# Autodesk Inventor assembly: Stadio8
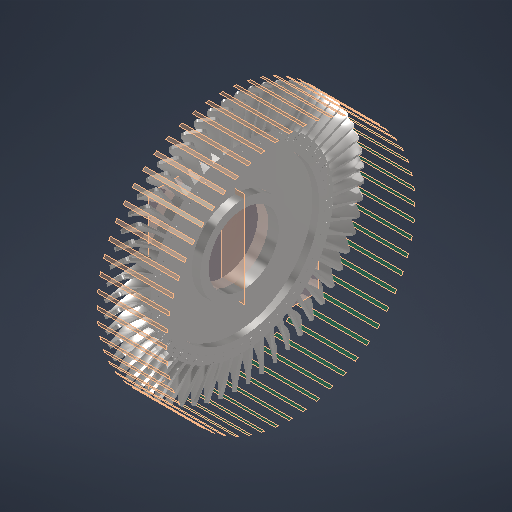
[picture p0: Inventor's stored thumbnail of the model, 512x512]
Saved by Autodesk Inventor 2026.2 (Build 302298010, 298A)
## iProperties
Created: 2026-04-24
Part Number: Stadio8
Document SubType Name: Assembly
Designer: Yan
Author: Yan
## Documents named in this file (3)
- C:\Users\Yan\Desktop\Turbina\Stadio8.iam
- C:\Users\Yan\Desktop\Turbina\DiscoPaleStadio8-DimensioniAprossimate.ipt
- C:\Users\Yan\Desktop\Turbina\PalaStadio8.ipt
## Components (57 placed, 2 different names)
1. DiscoPaleStadio8-DimensioniAprossimate:1 — Mate:1, Mate:2, Mate:3, Mate:4, Mate:5, Mate:6, Mate:7, Mate:8, Mate:9, Mate:10, Mate:11, Mate:12, Mate:13, Mate:14, Mate:15, Mate:16, Mate:17, Mate:18, Mate:19, Mate:20, Mate:21, Mate:22, Mate:23, Mate:24, Mate:25, Mate:26, Mate:27, Mate:28, Mate:29, Mate:30, Mate:31, Mate:32, Mate:33, Mate:34, Mate:35, Mate:36, Mate:37, Mate:38, Mate:39, Mate:40, Mate:41, Mate:42, Mate:43, Mate:44, Mate:45, Mate:46, Mate:47, Mate:48, Mate:49, Mate:50, Mate:51, Mate:52, Mate:53, Mate:54, Mate:55, Mate:56, Mate:57, Mate:58, Mate:59, Mate:60, Mate:62, Mate:63, Mate:64, Mate:65, Mate:66, Mate:67, Mate:68, Mate:69, Mate:70, Mate:71, Mate:72, Mate:73, Mate:74, Mate:75, Mate:76, Mate:77, Mate:78, Mate:79, Mate:80, Mate:81, Mate:82, Mate:83, Mate:84, Mate:85, Mate:86, Mate:87, Mate:88, Mate:89, Mate:90, Mate:91, Mate:92, Mate:93, Mate:94, Mate:95, Mate:96, Mate:97, Mate:98, Mate:99, Mate:100, Mate:101, Mate:102, Mate:103, Mate:104, Mate:105, Mate:106, Mate:107, Mate:108, Mate:109, Mate:110, Mate:111, Mate:112, Flush:1, Flush:2, Flush:3, Flush:4, Flush:5, Flush:6, Flush:7, Flush:8, Flush:9, Flush:10, Flush:11, Flush:12, Flush:13, Flush:14, Flush:15, Flush:16, Flush:17, Flush:18, Flush:19, Flush:20, Flush:21, Flush:22, Flush:23, Flush:24, Flush:25, Flush:26, Flush:27, Flush:28, Flush:29, Flush:30, Flush:31, Flush:32, Flush:33, Flush:34, Flush:35, Flush:36, Flush:37, Flush:38, Flush:39, Flush:40, Flush:41, Flush:42, Flush:43, Flush:44, Flush:45, Flush:46, Flush:47, Flush:48, Flush:49, Flush:50, Flush:51, Flush:52, Flush:53, Flush:54, Flush:55, Flush:56
2. PalaStadio8:1 — Mate:1, Mate:59, Flush:42
3. PalaStadio8:2 — Mate:2, Mate:58, Flush:43
4. PalaStadio8:3 — Mate:3, Mate:57, Flush:44
5. PalaStadio8:4 — Mate:4, Mate:56, Flush:45
6. PalaStadio8:5 — Mate:5, Mate:55, Flush:46
7. PalaStadio8:6 — Mate:6, Mate:54, Flush:47
8. PalaStadio8:7 — Mate:7, Mate:53, Flush:48
9. PalaStadio8:8 — Mate:8, Mate:52, Flush:49
10. PalaStadio8:9 — Mate:9, Mate:51, Flush:50
11. PalaStadio8:10 — Mate:10, Mate:50, Flush:51
12. PalaStadio8:11 — Mate:11, Mate:49, Flush:52
13. PalaStadio8:12 — Mate:12, Mate:48, Flush:53
14. PalaStadio8:13 — Mate:13, Mate:47, Flush:54
15. PalaStadio8:14 — Mate:14, Mate:46, Flush:55
16. PalaStadio8:15 — Mate:15, Mate:45, Flush:56
17. PalaStadio8:16 — Mate:16, Mate:44, Flush:2
18. PalaStadio8:17 — Mate:17, Mate:43, Flush:1
19. PalaStadio8:18 — Mate:18, Mate:42, Flush:3
20. PalaStadio8:19 — Mate:19, Mate:41, Flush:4
21. PalaStadio8:20 — Mate:20, Mate:40, Flush:5
22. PalaStadio8:21 — Mate:30, Mate:32, Flush:15
23. PalaStadio8:22 — Mate:29, Mate:31, Flush:14
24. PalaStadio8:23 — Mate:28, Mate:33, Flush:13
25. PalaStadio8:24 — Mate:27, Mate:60, Flush:12
26. PalaStadio8:25 — Mate:26, Mate:34, Flush:11
27. PalaStadio8:26 — Mate:25, Mate:35, Flush:10
28. PalaStadio8:27 — Mate:24, Mate:36, Flush:9
29. PalaStadio8:28 — Mate:23, Mate:37, Flush:8
30. PalaStadio8:29 — Mate:22, Mate:38, Flush:7
31. PalaStadio8:30 — Mate:21, Mate:39, Flush:6
32. PalaStadio8:31 — Mate:62, Mate:111, Flush:17
33. PalaStadio8:32 — Mate:64, Mate:112, Flush:18
34. PalaStadio8:33 — Mate:65, Mate:109, Flush:19
35. PalaStadio8:34 — Mate:66, Mate:108, Flush:20
36. PalaStadio8:35 — Mate:67, Mate:107, Flush:21
37. PalaStadio8:36 — Mate:68, Mate:106, Flush:22
38. PalaStadio8:37 — Mate:69, Mate:105, Flush:23
39. PalaStadio8:38 — Mate:70, Mate:104, Flush:24
40. PalaStadio8:39 — Mate:71, Mate:103, Flush:25
41. PalaStadio8:40 — Mate:63, Mate:110, Flush:16
42. PalaStadio8:41 — Mate:81, Mate:94, Flush:35
43. PalaStadio8:42 — Mate:80, Mate:95, Flush:34
44. PalaStadio8:43 — Mate:79, Mate:96, Flush:33
45. PalaStadio8:44 — Mate:78, Mate:97, Flush:32
46. PalaStadio8:45 — Mate:77, Mate:98, Flush:31
47. PalaStadio8:46 — Mate:76, Mate:99, Flush:30
48. PalaStadio8:47 — Mate:75, Mate:100, Flush:29
49. PalaStadio8:48 — Mate:74, Flush:28
50. PalaStadio8:49 — Mate:73, Mate:101, Flush:27
51. PalaStadio8:50 — Mate:72, Mate:102, Flush:26
52. PalaStadio8:51 — Mate:87, Mate:88, Flush:41
53. PalaStadio8:52 — Mate:86, Mate:89, Flush:40
54. PalaStadio8:53 — Mate:85, Mate:90, Flush:39
55. PalaStadio8:54 — Mate:84, Mate:91, Flush:38
56. PalaStadio8:55 — Mate:83, Mate:92, Flush:37
57. PalaStadio8:56 — Mate:82, Mate:93, Flush:36
## Relationships (167: Mate 111, Flush 56)
- Mate:1: DiscoPaleStadio8-DimensioniAprossimate:1 ↔ PalaStadio8:1
- Mate:2: DiscoPaleStadio8-DimensioniAprossimate:1 ↔ PalaStadio8:2
- Mate:3: DiscoPaleStadio8-DimensioniAprossimate:1 ↔ PalaStadio8:3
- Mate:4: DiscoPaleStadio8-DimensioniAprossimate:1 ↔ PalaStadio8:4
- Mate:5: DiscoPaleStadio8-DimensioniAprossimate:1 ↔ PalaStadio8:5
- Mate:6: DiscoPaleStadio8-DimensioniAprossimate:1 ↔ PalaStadio8:6
- Mate:7: DiscoPaleStadio8-DimensioniAprossimate:1 ↔ PalaStadio8:7
- Mate:8: DiscoPaleStadio8-DimensioniAprossimate:1 ↔ PalaStadio8:8
- Mate:9: DiscoPaleStadio8-DimensioniAprossimate:1 ↔ PalaStadio8:9
- Mate:10: DiscoPaleStadio8-DimensioniAprossimate:1 ↔ PalaStadio8:10
- Mate:11: DiscoPaleStadio8-DimensioniAprossimate:1 ↔ PalaStadio8:11
- Mate:12: DiscoPaleStadio8-DimensioniAprossimate:1 ↔ PalaStadio8:12
- Mate:13: DiscoPaleStadio8-DimensioniAprossimate:1 ↔ PalaStadio8:13
- Mate:14: DiscoPaleStadio8-DimensioniAprossimate:1 ↔ PalaStadio8:14
- Mate:15: DiscoPaleStadio8-DimensioniAprossimate:1 ↔ PalaStadio8:15
- Mate:16: DiscoPaleStadio8-DimensioniAprossimate:1 ↔ PalaStadio8:16
- Mate:17: DiscoPaleStadio8-DimensioniAprossimate:1 ↔ PalaStadio8:17
- Mate:18: DiscoPaleStadio8-DimensioniAprossimate:1 ↔ PalaStadio8:18
- Mate:19: DiscoPaleStadio8-DimensioniAprossimate:1 ↔ PalaStadio8:19
- Mate:20: DiscoPaleStadio8-DimensioniAprossimate:1 ↔ PalaStadio8:20
- Mate:21: DiscoPaleStadio8-DimensioniAprossimate:1 ↔ PalaStadio8:30
- Mate:22: DiscoPaleStadio8-DimensioniAprossimate:1 ↔ PalaStadio8:29
- Mate:23: DiscoPaleStadio8-DimensioniAprossimate:1 ↔ PalaStadio8:28
- Mate:24: DiscoPaleStadio8-DimensioniAprossimate:1 ↔ PalaStadio8:27
- Mate:25: DiscoPaleStadio8-DimensioniAprossimate:1 ↔ PalaStadio8:26
- Mate:26: DiscoPaleStadio8-DimensioniAprossimate:1 ↔ PalaStadio8:25
- Mate:27: DiscoPaleStadio8-DimensioniAprossimate:1 ↔ PalaStadio8:24
- Mate:28: DiscoPaleStadio8-DimensioniAprossimate:1 ↔ PalaStadio8:23
- Mate:29: DiscoPaleStadio8-DimensioniAprossimate:1 ↔ PalaStadio8:22
- Mate:30: DiscoPaleStadio8-DimensioniAprossimate:1 ↔ PalaStadio8:21
- Mate:31: DiscoPaleStadio8-DimensioniAprossimate:1 ↔ PalaStadio8:22
- Mate:32: DiscoPaleStadio8-DimensioniAprossimate:1 ↔ PalaStadio8:21
- Mate:33: DiscoPaleStadio8-DimensioniAprossimate:1 ↔ PalaStadio8:23
- Mate:34: DiscoPaleStadio8-DimensioniAprossimate:1 ↔ PalaStadio8:25
- Mate:35: DiscoPaleStadio8-DimensioniAprossimate:1 ↔ PalaStadio8:26
- Mate:36: DiscoPaleStadio8-DimensioniAprossimate:1 ↔ PalaStadio8:27
- Mate:37: DiscoPaleStadio8-DimensioniAprossimate:1 ↔ PalaStadio8:28
- Mate:38: DiscoPaleStadio8-DimensioniAprossimate:1 ↔ PalaStadio8:29
- Mate:39: DiscoPaleStadio8-DimensioniAprossimate:1 ↔ PalaStadio8:30
- Mate:40: DiscoPaleStadio8-DimensioniAprossimate:1 ↔ PalaStadio8:20
- Mate:41: DiscoPaleStadio8-DimensioniAprossimate:1 ↔ PalaStadio8:19
- Mate:42: DiscoPaleStadio8-DimensioniAprossimate:1 ↔ PalaStadio8:18
- Mate:43: DiscoPaleStadio8-DimensioniAprossimate:1 ↔ PalaStadio8:17
- Mate:44: DiscoPaleStadio8-DimensioniAprossimate:1 ↔ PalaStadio8:16
- Mate:45: DiscoPaleStadio8-DimensioniAprossimate:1 ↔ PalaStadio8:15
- Mate:46: DiscoPaleStadio8-DimensioniAprossimate:1 ↔ PalaStadio8:14
- Mate:47: DiscoPaleStadio8-DimensioniAprossimate:1 ↔ PalaStadio8:13
- Mate:48: DiscoPaleStadio8-DimensioniAprossimate:1 ↔ PalaStadio8:12
- Mate:49: DiscoPaleStadio8-DimensioniAprossimate:1 ↔ PalaStadio8:11
- Mate:50: DiscoPaleStadio8-DimensioniAprossimate:1 ↔ PalaStadio8:10
- Mate:51: DiscoPaleStadio8-DimensioniAprossimate:1 ↔ PalaStadio8:9
- Mate:52: DiscoPaleStadio8-DimensioniAprossimate:1 ↔ PalaStadio8:8
- Mate:53: DiscoPaleStadio8-DimensioniAprossimate:1 ↔ PalaStadio8:7
- Mate:54: DiscoPaleStadio8-DimensioniAprossimate:1 ↔ PalaStadio8:6
- Mate:55: DiscoPaleStadio8-DimensioniAprossimate:1 ↔ PalaStadio8:5
- Mate:56: DiscoPaleStadio8-DimensioniAprossimate:1 ↔ PalaStadio8:4
- Mate:57: DiscoPaleStadio8-DimensioniAprossimate:1 ↔ PalaStadio8:3
- Mate:58: DiscoPaleStadio8-DimensioniAprossimate:1 ↔ PalaStadio8:2
- Mate:59: DiscoPaleStadio8-DimensioniAprossimate:1 ↔ PalaStadio8:1
- Mate:60: DiscoPaleStadio8-DimensioniAprossimate:1 ↔ PalaStadio8:24
- Mate:62: DiscoPaleStadio8-DimensioniAprossimate:1 ↔ PalaStadio8:31
- Mate:63: DiscoPaleStadio8-DimensioniAprossimate:1 ↔ PalaStadio8:40
- Mate:64: DiscoPaleStadio8-DimensioniAprossimate:1 ↔ PalaStadio8:32
- Mate:65: DiscoPaleStadio8-DimensioniAprossimate:1 ↔ PalaStadio8:33
- Mate:66: DiscoPaleStadio8-DimensioniAprossimate:1 ↔ PalaStadio8:34
- Mate:67: DiscoPaleStadio8-DimensioniAprossimate:1 ↔ PalaStadio8:35
- Mate:68: DiscoPaleStadio8-DimensioniAprossimate:1 ↔ PalaStadio8:36
- Mate:69: DiscoPaleStadio8-DimensioniAprossimate:1 ↔ PalaStadio8:37
- Mate:70: DiscoPaleStadio8-DimensioniAprossimate:1 ↔ PalaStadio8:38
- Mate:71: DiscoPaleStadio8-DimensioniAprossimate:1 ↔ PalaStadio8:39
- Mate:72: DiscoPaleStadio8-DimensioniAprossimate:1 ↔ PalaStadio8:50
- Mate:73: DiscoPaleStadio8-DimensioniAprossimate:1 ↔ PalaStadio8:49
- Mate:74: DiscoPaleStadio8-DimensioniAprossimate:1 ↔ PalaStadio8:48
- Mate:75: DiscoPaleStadio8-DimensioniAprossimate:1 ↔ PalaStadio8:47
- Mate:76: DiscoPaleStadio8-DimensioniAprossimate:1 ↔ PalaStadio8:46
- Mate:77: DiscoPaleStadio8-DimensioniAprossimate:1 ↔ PalaStadio8:45
- Mate:78: DiscoPaleStadio8-DimensioniAprossimate:1 ↔ PalaStadio8:44
- Mate:79: DiscoPaleStadio8-DimensioniAprossimate:1 ↔ PalaStadio8:43
- Mate:80: DiscoPaleStadio8-DimensioniAprossimate:1 ↔ PalaStadio8:42
- Mate:81: DiscoPaleStadio8-DimensioniAprossimate:1 ↔ PalaStadio8:41
- Mate:82: DiscoPaleStadio8-DimensioniAprossimate:1 ↔ PalaStadio8:56
- Mate:83: DiscoPaleStadio8-DimensioniAprossimate:1 ↔ PalaStadio8:55
- Mate:84: DiscoPaleStadio8-DimensioniAprossimate:1 ↔ PalaStadio8:54
- Mate:85: DiscoPaleStadio8-DimensioniAprossimate:1 ↔ PalaStadio8:53
- Mate:86: DiscoPaleStadio8-DimensioniAprossimate:1 ↔ PalaStadio8:52
- Mate:87: DiscoPaleStadio8-DimensioniAprossimate:1 ↔ PalaStadio8:51
- Mate:88: DiscoPaleStadio8-DimensioniAprossimate:1 ↔ PalaStadio8:51
- Mate:89: DiscoPaleStadio8-DimensioniAprossimate:1 ↔ PalaStadio8:52
- Mate:90: DiscoPaleStadio8-DimensioniAprossimate:1 ↔ PalaStadio8:53
- Mate:91: DiscoPaleStadio8-DimensioniAprossimate:1 ↔ PalaStadio8:54
- Mate:92: DiscoPaleStadio8-DimensioniAprossimate:1 ↔ PalaStadio8:55
- Mate:93: DiscoPaleStadio8-DimensioniAprossimate:1 ↔ PalaStadio8:56
- Mate:94: DiscoPaleStadio8-DimensioniAprossimate:1 ↔ PalaStadio8:41
- Mate:95: DiscoPaleStadio8-DimensioniAprossimate:1 ↔ PalaStadio8:42
- Mate:96: DiscoPaleStadio8-DimensioniAprossimate:1 ↔ PalaStadio8:43
- Mate:97: DiscoPaleStadio8-DimensioniAprossimate:1 ↔ PalaStadio8:44
- Mate:98: DiscoPaleStadio8-DimensioniAprossimate:1 ↔ PalaStadio8:45
- Mate:99: DiscoPaleStadio8-DimensioniAprossimate:1 ↔ PalaStadio8:46
- Mate:100: DiscoPaleStadio8-DimensioniAprossimate:1 ↔ PalaStadio8:47
- Mate:101: DiscoPaleStadio8-DimensioniAprossimate:1 ↔ PalaStadio8:49
- Mate:102: DiscoPaleStadio8-DimensioniAprossimate:1 ↔ PalaStadio8:50
- Mate:103: DiscoPaleStadio8-DimensioniAprossimate:1 ↔ PalaStadio8:39
- Mate:104: DiscoPaleStadio8-DimensioniAprossimate:1 ↔ PalaStadio8:38
- Mate:105: DiscoPaleStadio8-DimensioniAprossimate:1 ↔ PalaStadio8:37
- Mate:106: DiscoPaleStadio8-DimensioniAprossimate:1 ↔ PalaStadio8:36
- Mate:107: DiscoPaleStadio8-DimensioniAprossimate:1 ↔ PalaStadio8:35
- Mate:108: DiscoPaleStadio8-DimensioniAprossimate:1 ↔ PalaStadio8:34
- Mate:109: DiscoPaleStadio8-DimensioniAprossimate:1 ↔ PalaStadio8:33
- Mate:110: DiscoPaleStadio8-DimensioniAprossimate:1 ↔ PalaStadio8:40
- Mate:111: DiscoPaleStadio8-DimensioniAprossimate:1 ↔ PalaStadio8:31
- Mate:112: DiscoPaleStadio8-DimensioniAprossimate:1 ↔ PalaStadio8:32
- Flush:1: DiscoPaleStadio8-DimensioniAprossimate:1 ↔ PalaStadio8:17
- Flush:2: DiscoPaleStadio8-DimensioniAprossimate:1 ↔ PalaStadio8:16
- Flush:3: DiscoPaleStadio8-DimensioniAprossimate:1 ↔ PalaStadio8:18
- Flush:4: DiscoPaleStadio8-DimensioniAprossimate:1 ↔ PalaStadio8:19
- Flush:5: DiscoPaleStadio8-DimensioniAprossimate:1 ↔ PalaStadio8:20
- Flush:6: DiscoPaleStadio8-DimensioniAprossimate:1 ↔ PalaStadio8:30
- Flush:7: DiscoPaleStadio8-DimensioniAprossimate:1 ↔ PalaStadio8:29
- Flush:8: DiscoPaleStadio8-DimensioniAprossimate:1 ↔ PalaStadio8:28
- Flush:9: DiscoPaleStadio8-DimensioniAprossimate:1 ↔ PalaStadio8:27
- Flush:10: DiscoPaleStadio8-DimensioniAprossimate:1 ↔ PalaStadio8:26
- Flush:11: DiscoPaleStadio8-DimensioniAprossimate:1 ↔ PalaStadio8:25
- Flush:12: DiscoPaleStadio8-DimensioniAprossimate:1 ↔ PalaStadio8:24
- Flush:13: DiscoPaleStadio8-DimensioniAprossimate:1 ↔ PalaStadio8:23
- Flush:14: DiscoPaleStadio8-DimensioniAprossimate:1 ↔ PalaStadio8:22
- Flush:15: DiscoPaleStadio8-DimensioniAprossimate:1 ↔ PalaStadio8:21
- Flush:16: DiscoPaleStadio8-DimensioniAprossimate:1 ↔ PalaStadio8:40
- Flush:17: DiscoPaleStadio8-DimensioniAprossimate:1 ↔ PalaStadio8:31
- Flush:18: DiscoPaleStadio8-DimensioniAprossimate:1 ↔ PalaStadio8:32
- Flush:19: DiscoPaleStadio8-DimensioniAprossimate:1 ↔ PalaStadio8:33
- Flush:20: DiscoPaleStadio8-DimensioniAprossimate:1 ↔ PalaStadio8:34
- Flush:21: DiscoPaleStadio8-DimensioniAprossimate:1 ↔ PalaStadio8:35
- Flush:22: DiscoPaleStadio8-DimensioniAprossimate:1 ↔ PalaStadio8:36
- Flush:23: DiscoPaleStadio8-DimensioniAprossimate:1 ↔ PalaStadio8:37
- Flush:24: DiscoPaleStadio8-DimensioniAprossimate:1 ↔ PalaStadio8:38
- Flush:25: DiscoPaleStadio8-DimensioniAprossimate:1 ↔ PalaStadio8:39
- Flush:26: DiscoPaleStadio8-DimensioniAprossimate:1 ↔ PalaStadio8:50
- Flush:27: DiscoPaleStadio8-DimensioniAprossimate:1 ↔ PalaStadio8:49
- Flush:28: DiscoPaleStadio8-DimensioniAprossimate:1 ↔ PalaStadio8:48
- Flush:29: DiscoPaleStadio8-DimensioniAprossimate:1 ↔ PalaStadio8:47
- Flush:30: DiscoPaleStadio8-DimensioniAprossimate:1 ↔ PalaStadio8:46
- Flush:31: DiscoPaleStadio8-DimensioniAprossimate:1 ↔ PalaStadio8:45
- Flush:32: DiscoPaleStadio8-DimensioniAprossimate:1 ↔ PalaStadio8:44
- Flush:33: DiscoPaleStadio8-DimensioniAprossimate:1 ↔ PalaStadio8:43
- Flush:34: DiscoPaleStadio8-DimensioniAprossimate:1 ↔ PalaStadio8:42
- Flush:35: DiscoPaleStadio8-DimensioniAprossimate:1 ↔ PalaStadio8:41
- Flush:36: DiscoPaleStadio8-DimensioniAprossimate:1 ↔ PalaStadio8:56
- Flush:37: DiscoPaleStadio8-DimensioniAprossimate:1 ↔ PalaStadio8:55
- Flush:38: DiscoPaleStadio8-DimensioniAprossimate:1 ↔ PalaStadio8:54
- Flush:39: DiscoPaleStadio8-DimensioniAprossimate:1 ↔ PalaStadio8:53
- Flush:40: DiscoPaleStadio8-DimensioniAprossimate:1 ↔ PalaStadio8:52
- Flush:41: DiscoPaleStadio8-DimensioniAprossimate:1 ↔ PalaStadio8:51
- Flush:42: DiscoPaleStadio8-DimensioniAprossimate:1 ↔ PalaStadio8:1
- Flush:43: DiscoPaleStadio8-DimensioniAprossimate:1 ↔ PalaStadio8:2
- Flush:44: DiscoPaleStadio8-DimensioniAprossimate:1 ↔ PalaStadio8:3
- Flush:45: DiscoPaleStadio8-DimensioniAprossimate:1 ↔ PalaStadio8:4
- Flush:46: DiscoPaleStadio8-DimensioniAprossimate:1 ↔ PalaStadio8:5
- Flush:47: DiscoPaleStadio8-DimensioniAprossimate:1 ↔ PalaStadio8:6
- Flush:48: DiscoPaleStadio8-DimensioniAprossimate:1 ↔ PalaStadio8:7
- Flush:49: DiscoPaleStadio8-DimensioniAprossimate:1 ↔ PalaStadio8:8
- Flush:50: DiscoPaleStadio8-DimensioniAprossimate:1 ↔ PalaStadio8:9
- Flush:51: DiscoPaleStadio8-DimensioniAprossimate:1 ↔ PalaStadio8:10
- Flush:52: DiscoPaleStadio8-DimensioniAprossimate:1 ↔ PalaStadio8:11
- Flush:53: DiscoPaleStadio8-DimensioniAprossimate:1 ↔ PalaStadio8:12
- Flush:54: DiscoPaleStadio8-DimensioniAprossimate:1 ↔ PalaStadio8:13
- Flush:55: DiscoPaleStadio8-DimensioniAprossimate:1 ↔ PalaStadio8:14
- Flush:56: DiscoPaleStadio8-DimensioniAprossimate:1 ↔ PalaStadio8:15
